# Autodesk Inventor assembly: CHIP_EXTRACTION_EXAMPLE
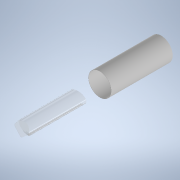
[picture p0: Inventor's stored thumbnail of the model, 180x180]
Saved by Autodesk Inventor 2022 (Build 260153070, 153G)
## iProperties
Created: 2022-04-03
Part Number: CHIP_EXTRACTION_EXAMPLE
Document SubType Name: Assembly
Designer: a laptop
Author: a laptop
## Documents named in this file (3)
- C:\Users\a laptop\Desktop\CADTable_2022_Project\CHIP_EXTRACTION_EXAMPLE.iam
- C:\Users\a laptop\Desktop\CADTable_2022_Project\chip_holder_EXTRACTOR.ipt
- C:\Users\a laptop\Desktop\CADTable_2022_Project\REF_CAN.ipt
## Components (2 placed, 2 different names)
1. chip_holder_EXTRACTOR:1 — Mate:1, Angle:1
2. REF_CAN:1 — Mate:1, Angle:1
## Relationships (2: Mate 1, Angle 1)
- Mate:1: chip_holder_EXTRACTOR:1 ↔ REF_CAN:1
- Angle:1 (0 deg): chip_holder_EXTRACTOR:1 ↔ REF_CAN:1
